# Autodesk Inventor assembly: gate_valve_assembly
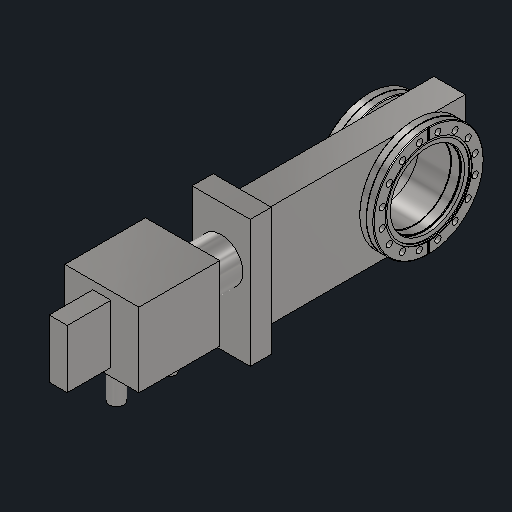
[picture p0: Inventor's stored thumbnail of the model, 512x512]
Saved by Autodesk Inventor 2027.1 (Build 311270010, 270A)
## iProperties
Created: 2026-03-12
Part Number: gate_valve_assembly
Document SubType Name: Assembly
Designer: zetsu
Author: zetsu
## Documents named in this file (4)
- C:\Users\queezz\Dropbox\Drawings\pihti-cad\Plasma Vessel_2026\gate_valve\CF150-gatevalve-assembly.iam
- C:\Users\queezz\Dropbox\Drawings\pihti-cad\Plasma Vessel_2026\gate_valve\CF150-gatevalve-body.ipt
- C:\Users\queezz\Dropbox\Drawings\pihti-cad\Plasma Vessel\Plasma-vacuum-cross\UFC-152.ipt
- C:\Users\queezz\Dropbox\Drawings\pihti-cad\Plasma Vessel\Plasma-vacuum-cross\UFC.ipt
## Components (3 placed, 2 different names)
1. CF150-gatevalve-body:1 — Mate:1, Mate:2, Mate:3, Mate:4, Angle:1, Angle:2
2. UFC-152:1 — Mate:2, Mate:4, Angle:2
3. UFC-152:2 — Mate:1, Mate:3, Angle:1
## Relationships (6: Mate 4, Angle 2)
- Mate:1: CF150-gatevalve-body:1 ↔ UFC-152:2
- Mate:2: CF150-gatevalve-body:1 ↔ UFC-152:1
- Mate:3: CF150-gatevalve-body:1 ↔ UFC-152:2
- Mate:4: CF150-gatevalve-body:1 ↔ UFC-152:1
- Angle:1 (0 deg): CF150-gatevalve-body:1 ↔ UFC-152:2
- Angle:2 (0 deg): CF150-gatevalve-body:1 ↔ UFC-152:1
